# Autodesk Inventor assembly: WJ_75
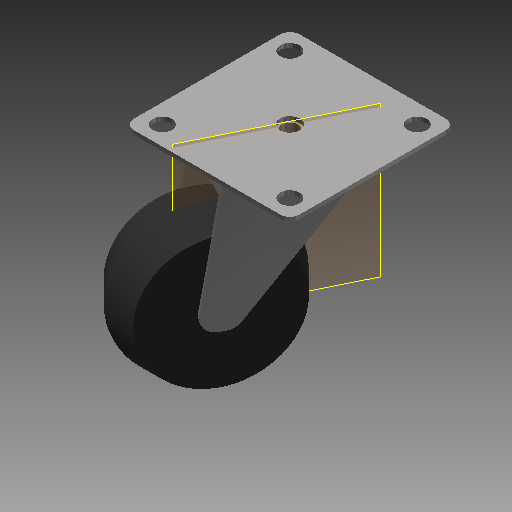
[picture p0: Inventor's stored thumbnail of the model, 512x512]
Saved by Autodesk Inventor 2019 (Build 230136000, 136)
## iProperties
Created: 2019-04-26
Part Number: WJ_75
Material: 일반
Document SubType Name: Assembly
Designer: hinmo
Author: hinmo
## Documents named in this file (4)
- C:\Users\hinmo\Documents\Inventor\Projects\2019_CapstoneDesign\WJ_75.iam
- C:\Users\hinmo\Documents\Inventor\Projects\2019_CapstoneDesign\Part_Metal.ipt
- C:\Users\hinmo\Documents\Inventor\Projects\2019_CapstoneDesign\Part_MetalLeg.ipt
- C:\Users\hinmo\Documents\Inventor\Projects\2019_CapstoneDesign\Part_Rubber.ipt
## Components (3 placed, 3 different names)
1. Part_Metal:1 — 메이트:1, 메이트:2
2. Part_MetalLeg:1 — 메이트:1, 메이트:2, 메이트:3, 메이트:4
3. Part_Rubber:1 — 메이트:3, 메이트:4
## Relationships (4: Mate 4)
- 메이트:1 [Mate]: Part_Metal:1 ↔ Part_MetalLeg:1
- 메이트:2 [Mate]: Part_Metal:1 ↔ Part_MetalLeg:1
- 메이트:3 [Mate]: Part_MetalLeg:1 ↔ Part_Rubber:1
- 메이트:4 [Mate]: Part_MetalLeg:1 ↔ Part_Rubber:1
